# Autodesk Inventor assembly: Assembly
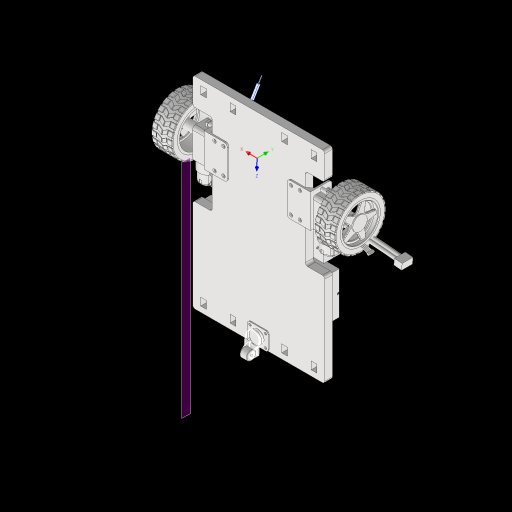
[picture p0: Inventor's stored thumbnail of the model, 512x512]
Saved by Autodesk Inventor 2024.3 (Build 283343010, 343A)
## iProperties
Created: 2025-04-09
Part Number: Assembly
Document SubType Name: Assembly
Designer: Oleg Kelner
Author: Oleg Kelner
## Documents named in this file (11)
- D:\Study\Prototyping\Assembly.iam
- D:\Work\HSHL\Kart\Kart Assembly Parts\chassis.ipt
- D:\Work\HSHL\Kart\Kart Assembly Parts\motor-with-tire.ipt
- D:\Study\Prototyping\motorHolder_MIR.ipt
- D:\Work\HSHL\Kart\Kart Assembly Parts\front-wheel.ipt
- D:\Work\HSHL\Kart\Kart Assembly Parts\motor-with-tire_MIR.ipt
- D:\Study\Prototyping\motorHolder_MIR_MIR.ipt
- D:\Work\HSHL\Kart\Kart Assembly Parts\lipo-battery.ipt
- D:\Work\HSHL\Kart\Kart Assembly Parts\arduino.ipt
- D:\Work\HSHL\Kart\Kart Assembly Parts\breadboard.ipt
- D:\Work\HSHL\Kart\Kart Assembly Parts\motorcontroler.ipt
## Components (10 placed, 10 different names)
1. chassis:1 — Angle:1, Planar:2, Mate:1, Mate:2, Flush:1, Mate:3, Mate:4, Mate:5, Rigid:1, Planar:3, Angle:2, Planar:4, Angle:3, Planar:5, Angle:4, Planar:6
2. motor-with-tire:1 — Rotational:4, Tangent:1, Rotational:5
3. motorHolder_MIR:1 — Rotational:4, Rotational:5, Planar:2, Mate:1, Mate:2
4. front-wheel:1 — Rigid:1
5. motor-with-tire_MIR:1 — Tangent:3, Rotational:6, Rotational:7
6. motorHolder_MIR_MIR:1 — Rotational:6, Rotational:7, Mate:3, Mate:4, Mate:5
7. lipo-battery:1 — Planar:3, Angle:2
8. arduino:1 — Planar:5, Angle:4
9. breadboard:1 — Planar:4, Angle:3
10. motorcontroler:1 — Planar:6
## Relationships (22: PlanarJoint 5, Mate 5, RevoluteJoint 4, Angle 4, Tangent 2, Flush 1, WeldJoint 1)
- Rotational:4 [RevoluteJoint]: motor-with-tire:1 ↔ motorHolder_MIR:1
- Angle:1 (0 deg): chassis:1
- Tangent:1: motor-with-tire:1
- Rotational:5 [RevoluteJoint]: motor-with-tire:1 ↔ motorHolder_MIR:1
- Planar:2: chassis:1 ↔ motorHolder_MIR:1
- Mate:1 (-21.5 mm): chassis:1 ↔ motorHolder_MIR:1
- Mate:2 (18 mm): chassis:1 ↔ motorHolder_MIR:1
- Flush:1 (-85 mm): chassis:1
- Tangent:3: motor-with-tire_MIR:1
- Rotational:6 [RevoluteJoint]: motor-with-tire_MIR:1 ↔ motorHolder_MIR_MIR:1
- Rotational:7 [RevoluteJoint]: motor-with-tire_MIR:1 ↔ motorHolder_MIR_MIR:1
- Mate:3 (-21.5 mm): chassis:1 ↔ motorHolder_MIR_MIR:1
- Mate:4 (18 mm): chassis:1 ↔ motorHolder_MIR_MIR:1
- Mate:5: chassis:1 ↔ motorHolder_MIR_MIR:1
- Rigid:1 [WeldJoint]: chassis:1 ↔ front-wheel:1
- Planar:3: chassis:1 ↔ lipo-battery:1
- Angle:2 (0 deg): chassis:1 ↔ lipo-battery:1
- Planar:4: chassis:1 ↔ breadboard:1
- Angle:3 (0 deg): chassis:1 ↔ breadboard:1
- Planar:5: chassis:1 ↔ arduino:1
- Angle:4 (0 deg): chassis:1 ↔ arduino:1
- Planar:6: chassis:1 ↔ motorcontroler:1
